# Autodesk Inventor assembly: b1
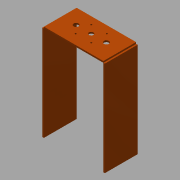
[picture p0: Inventor's stored thumbnail of the model, 180x180]
Saved by Autodesk Inventor 2016 (Build 200138000, 138)
## iProperties
Created: 2015-10-11
Part Number: b1
Document SubType Name: Assembly
Designer: daniel
Author: daniel
## Documents named in this file (3)
- C:\Users\daniel\Documents\GitHub\cardboard-stage-metric\stage\b1.iam
- C:\Users\daniel\Documents\GitHub\cardboard-stage-metric\stage\b1a.ipt
- C:\Users\daniel\Documents\GitHub\cardboard-stage-metric\stage\b1b.ipt
## Components (3 placed, 2 different names)
1. b1a:1 — Flush:2, Flush:3, Mate:1, Mate:2, Mate:3
2. b1b:1 — Flush:1, Flush:3, Mate:3
3. b1b:2 — Flush:1, Flush:2, Mate:1, Mate:2
## Relationships (6: Flush 3, Mate 3)
- Flush:1: b1b:1 ↔ b1b:2
- Flush:2: b1a:1 ↔ b1b:2
- Flush:3: b1a:1 ↔ b1b:1
- Mate:1: b1a:1 ↔ b1b:2
- Mate:2: b1a:1 ↔ b1b:2
- Mate:3: b1a:1 ↔ b1b:1
